# Autodesk Inventor assembly: Components dosplay
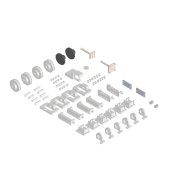
[picture p0: Inventor's stored thumbnail of the model, 180x180]
Saved by Autodesk Inventor 2020 (Build 240168000, 168)
## iProperties
Created: 2021-09-07
Part Number: Components dosplay
Document SubType Name: Assembly
Designer: ferrerx
Author: ferrerx
## Documents named in this file (17)
- C:\Users\ferrerx\Desktop\Projects\Prieto-Godino Lab\Drosophila Larvae Behavioural Device\Device design V3\Inventor Assembly\Components dosplay.iam
- C:\Users\ferrerx\Desktop\Projects\Prieto-Godino Lab\Drosophila Larvae Behavioural Device\Device design V3\Inventor Assembly\Arena spacer.ipt
- C:\Users\ferrerx\Desktop\Projects\Prieto-Godino Lab\Drosophila Larvae Behavioural Device\Device design V3\Inventor Assembly\Big pulley.ipt
- C:\Users\ferrerx\Desktop\Projects\Prieto-Godino Lab\Drosophila Larvae Behavioural Device\Device design V3\Inventor Assembly\Cart.ipt
- C:\Users\ferrerx\Desktop\Projects\Prieto-Godino Lab\Drosophila Larvae Behavioural Device\Device design V3\Inventor Assembly\cart_spacer.ipt
- C:\Users\ferrerx\Desktop\Projects\Prieto-Godino Lab\Drosophila Larvae Behavioural Device\Device design V3\Inventor Assembly\ISO - Spur gear 1M 20T 20PA 5FW ---S20A75H50L5.0N.ipt
- C:\Users\ferrerx\Desktop\Projects\Prieto-Godino Lab\Drosophila Larvae Behavioural Device\Device design V3\Inventor Assembly\ISO - Rack-spur - rectangular 1M 20PA 5FW 5PH 125L---SAll.ipt
- C:\Users\ferrerx\Desktop\Projects\Prieto-Godino Lab\Drosophila Larvae Behavioural Device\Device design V3\Inventor Assembly\Lead screw manual adjuster.ipt
- C:\Users\ferrerx\Desktop\Projects\Prieto-Godino Lab\Drosophila Larvae Behavioural Device\Device design V3\Inventor Assembly\LED linear array holder.ipt
- C:\Users\ferrerx\Desktop\Projects\Prieto-Godino Lab\Drosophila Larvae Behavioural Device\Device design V3\Inventor Assembly\LED Matrix 8X8 - attachment.ipt
- C:\Users\ferrerx\Desktop\Projects\Prieto-Godino Lab\Drosophila Larvae Behavioural Device\Device design V3\Inventor Assembly\Linear actuator servo attachment.ipt
- C:\Users\ferrerx\Desktop\Projects\Prieto-Godino Lab\Drosophila Larvae Behavioural Device\Device design V3\Inventor Assembly\M6 spacer.ipt
- C:\Users\ferrerx\Desktop\Projects\Prieto-Godino Lab\Drosophila Larvae Behavioural Device\Device design V3\Inventor Assembly\Micro servo holder.ipt
- C:\Users\ferrerx\Desktop\Projects\Prieto-Godino Lab\Drosophila Larvae Behavioural Device\Device design V3\Inventor Assembly\Raspberry pi HQ camera.ipt
- C:\Users\ferrerx\Desktop\Projects\Prieto-Godino Lab\Drosophila Larvae Behavioural Device\Device design V3\Inventor Assembly\Shaft atachment.ipt
- C:\Users\ferrerx\Desktop\Projects\Prieto-Godino Lab\Drosophila Larvae Behavioural Device\Device design V3\Inventor Assembly\Ultrasonic sensor holder.ipt
- C:\Users\ferrerx\Desktop\Projects\Prieto-Godino Lab\Drosophila Larvae Behavioural Device\Device design V3\Inventor Assembly\Belt tensor2.ipt
## Components (72 placed, 16 different names)
1. Arena spacer:1 — Mate:4
2. Arena spacer:2 — Mate:5
3. Arena spacer:3 — Mate:6
4. Arena spacer:4 — Mate:7
5. Arena spacer:5 — Mate:4
6. Arena spacer:6 — Mate:5, Tangent:1
7. Arena spacer:7 — Mate:6, Mate:52
8. Arena spacer:8 — Mate:7, Mate:53
9. Big pulley:1 — Mate:2, Mate:3
10. Big pulley:2 — Mate:1, Mate:2
11. Big pulley:3 — Mate:1
12. Big pulley:4 — Mate:3
13. Cart:1 — Flush:1, Mate:8
14. Cart:2 — Flush:1, Mate:8, Mate:9, Flush:2
15. Cart:3 — Mate:9, Flush:2, Flush:3, Mate:10
16. Cart:4 — Flush:3, Mate:10, Mate:17
17. cart_spacer:1 — Mate:12
18. cart_spacer:2 — Mate:11, Mate:12, Mate:13
19. cart_spacer:3 — Mate:11
20. cart_spacer:4 — Mate:13
21. cart_spacer:5 — Mate:14, Flush:17
22. cart_spacer:6 — Mate:14, Mate:15, Mate:16
23. cart_spacer:7 — Mate:15
24. cart_spacer:8 — Mate:16
25. cart_spacer:9 — Mate:21, Flush:17, Flush:18
26. cart_spacer:10 — Mate:21, Mate:22, Mate:23
27. cart_spacer:11 — Mate:22
28. cart_spacer:12 — Mate:23
29. cart_spacer:13 — Mate:24, Flush:18
30. cart_spacer:14 — Mate:24, Mate:25
31. cart_spacer:15 — Mate:25, Mate:26
32. cart_spacer:16 — Mate:26
33. ISO - Spur gear 1M 20T 20PA 5FW ---S20A75H50L5.0N:1 — Mate:27
34. ISO - Rack-spur - rectangular 1M 20PA 5FW 5PH 125L---SAll:1
35. Lead screw manual adjuster:1 — Mate:47
36. Lead screw manual adjuster:2 — Mate:47
37. LED linear array holder:1 — Flush:20, Flush:21, Flush:22, Flush:23, Flush:25
38. LED linear array holder:2 — Flush:20, Mate:46, Flush:24
39. LED linear array holder:3 — Flush:21, Flush:23, Flush:24
40. LED linear array holder:4 — Flush:22, Flush:25
41. LED Matrix 8X8 - attachment:1 — Mate:48
42. LED Matrix 8X8 - attachment:2 — Mate:49
43. Linear actuator servo attachment:1 — Flush:4
44. M6 spacer:1 — Mate:28, Mate:29, Mate:30, Mate:31
45. M6 spacer:2 — Mate:33, Mate:34, Mate:35, Mate:36
46. M6 spacer:3 — Mate:28
47. M6 spacer:4 — Mate:33
48. M6 spacer:5 — Mate:29
49. M6 spacer:6 — Mate:34
50. M6 spacer:7 — Mate:30, Mate:32
51. M6 spacer:8 — Mate:35
52. M6 spacer:9 — Mate:31
53. M6 spacer:10 — Mate:36, Mate:37
54. M6 spacer:11 — Mate:32
55. M6 spacer:12 — Mate:37
56. Micro servo holder:1 — Flush:5, Flush:6, Flush:7, Flush:8, Mate:18, Flush:10
57. Micro servo holder:2 — Flush:5, Flush:9, Flush:14
58. Micro servo holder:3 — Flush:6, Flush:13
59. Micro servo holder:4 — Flush:7, Flush:12
60. Micro servo holder:5 — Flush:8, Flush:11, Flush:13, Flush:14
61. Micro servo holder:6 — Flush:9, Flush:10, Flush:11, Flush:12
62. Raspberry pi HQ camera:1
63. Shaft atachment:1 — Mate:19, Mate:20, Flush:16, Mate:42
64. Shaft atachment:2 — Mate:20, Flush:16, Mate:44
65. Shaft atachment:3 — Mate:38, Mate:42, Mate:43
66. Shaft atachment:4 — Mate:39, Mate:43
67. Shaft atachment:5 — Mate:40, Mate:44, Mate:45
68. Shaft atachment:6 — Mate:41, Mate:45
69. Ultrasonic sensor holder:1 — Flush:19, Mate:50
70. Ultrasonic sensor holder:2 — Flush:19, Mate:51
71. Belt tensor2:1 — Flush:15
72. Belt tensor2:2 — Flush:15
## Relationships (79: Mate 53, Flush 25, Tangent 1)
- Mate:1: Big pulley:2 ↔ Big pulley:3
- Mate:2: Big pulley:1 ↔ Big pulley:2
- Mate:3: Big pulley:1 ↔ Big pulley:4
- Mate:4: Arena spacer:1 ↔ Arena spacer:5
- Mate:5: Arena spacer:2 ↔ Arena spacer:6
- Mate:6: Arena spacer:3 ↔ Arena spacer:7
- Mate:7: Arena spacer:4 ↔ Arena spacer:8
- Flush:1: Cart:1 ↔ Cart:2
- Mate:8: Cart:1 ↔ Cart:2
- Mate:9: Cart:2 ↔ Cart:3
- Flush:2: Cart:2 ↔ Cart:3
- Flush:3: Cart:3 ↔ Cart:4
- Mate:10: Cart:3 ↔ Cart:4
- Mate:11: cart_spacer:2 ↔ cart_spacer:3
- Mate:12: cart_spacer:1 ↔ cart_spacer:2
- Mate:13: cart_spacer:2 ↔ cart_spacer:4
- Mate:14: cart_spacer:5 ↔ cart_spacer:6
- Mate:15: cart_spacer:6 ↔ cart_spacer:7
- Mate:16: cart_spacer:6 ↔ cart_spacer:8
- Mate:17: Cart:4
- Flush:4: Linear actuator servo attachment:1
- Flush:5: Micro servo holder:1 ↔ Micro servo holder:2
- Flush:6: Micro servo holder:1 ↔ Micro servo holder:3
- Flush:7: Micro servo holder:1 ↔ Micro servo holder:4
- Flush:8: Micro servo holder:1 ↔ Micro servo holder:5
- Flush:9: Micro servo holder:2 ↔ Micro servo holder:6
- Mate:18: Micro servo holder:1
- Mate:19: Shaft atachment:1
- Flush:10: Micro servo holder:1 ↔ Micro servo holder:6
- Flush:11: Micro servo holder:5 ↔ Micro servo holder:6
- Flush:12: Micro servo holder:4 ↔ Micro servo holder:6
- Flush:13: Micro servo holder:3 ↔ Micro servo holder:5
- Flush:14: Micro servo holder:2 ↔ Micro servo holder:5
- Flush:15: Belt tensor2:1 ↔ Belt tensor2:2
- Mate:20: Shaft atachment:1 ↔ Shaft atachment:2
- Flush:16: Shaft atachment:1 ↔ Shaft atachment:2
- Mate:21: cart_spacer:9 ↔ cart_spacer:10
- Mate:22: cart_spacer:10 ↔ cart_spacer:11
- Mate:23: cart_spacer:10 ↔ cart_spacer:12
- Flush:17: cart_spacer:5 ↔ cart_spacer:9
- Mate:24: cart_spacer:13 ↔ cart_spacer:14
- Flush:18: cart_spacer:9 ↔ cart_spacer:13
- Mate:25: cart_spacer:14 ↔ cart_spacer:15
- Mate:26: cart_spacer:15 ↔ cart_spacer:16
- Mate:27: ISO - Spur gear 1M 20T 20PA 5FW ---S20A75H50L5.0N:1
- Mate:28: M6 spacer:1 ↔ M6 spacer:3
- Mate:29: M6 spacer:1 ↔ M6 spacer:5
- Mate:30: M6 spacer:1 ↔ M6 spacer:7
- Mate:31: M6 spacer:1 ↔ M6 spacer:9
- Mate:32: M6 spacer:7 ↔ M6 spacer:11
- Mate:33: M6 spacer:2 ↔ M6 spacer:4
- Mate:34: M6 spacer:2 ↔ M6 spacer:6
- Mate:35: M6 spacer:2 ↔ M6 spacer:8
- Mate:36: M6 spacer:2 ↔ M6 spacer:10
- Mate:37: M6 spacer:10 ↔ M6 spacer:12
- Flush:19: Ultrasonic sensor holder:1 ↔ Ultrasonic sensor holder:2
- Mate:38: Shaft atachment:3
- Mate:39: Shaft atachment:4
- Mate:40: Shaft atachment:5
- Mate:41: Shaft atachment:6
- Mate:42: Shaft atachment:1 ↔ Shaft atachment:3
- Mate:43: Shaft atachment:3 ↔ Shaft atachment:4
- Mate:44: Shaft atachment:2 ↔ Shaft atachment:5
- Mate:45: Shaft atachment:5 ↔ Shaft atachment:6
- Flush:20: LED linear array holder:1 ↔ LED linear array holder:2
- Mate:46: LED linear array holder:2
- Flush:21: LED linear array holder:1 ↔ LED linear array holder:3
- Flush:22: LED linear array holder:1 ↔ LED linear array holder:4
- Flush:23: LED linear array holder:1 ↔ LED linear array holder:3
- Flush:24: LED linear array holder:2 ↔ LED linear array holder:3
- Flush:25: LED linear array holder:1 ↔ LED linear array holder:4
- Mate:47: Lead screw manual adjuster:1 ↔ Lead screw manual adjuster:2
- Mate:48: LED Matrix 8X8 - attachment:1
- Mate:49: LED Matrix 8X8 - attachment:2
- Mate:50: Ultrasonic sensor holder:1
- Mate:51: Ultrasonic sensor holder:2
- Tangent:1: Arena spacer:6
- Mate:52: Arena spacer:7
- Mate:53: Arena spacer:8
